# Autodesk Inventor assembly: Gearbox - 54 to 1
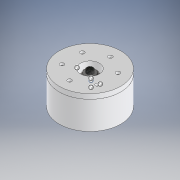
[picture p0: Inventor's stored thumbnail of the model, 180x180]
Saved by Autodesk Inventor 2017 SP1 (Build 210196100, 196)
## iProperties
Created: 2017-09-22
Part Number: Gearbox - 54 to 1
Document SubType Name: Assembly
Designer: Zach
Author: Zach
## Documents named in this file (9)
- C:\Users\Zach\Documents\GitHub\tr1\lib\Gearbox 8;1\Gearbox 8;1.iam
- C:\Users\Zach\Documents\GitHub\tr1\lib\Gearbox 8;1\Base.ipt
- C:\Users\Zach\Documents\GitHub\tr1\lib\22x8x8mm Bearing.ipt
- C:\Users\Zach\Documents\GitHub\tr1\lib\Gearbox 8;1\3mm Brass Rod.ipt
- C:\Users\Zach\Documents\GitHub\tr1\lib\CNS 3129 - M 8 x 1.25.ipt
- C:\Users\Zach\Documents\GitHub\tr1\lib\Gearbox 8;1\GearSet 1.iam
- C:\Users\Zach\Documents\GitHub\tr1\lib\Gearbox 8;1\Small Gear.ipt
- C:\Users\Zach\Documents\GitHub\tr1\lib\Gearbox 8;1\Cover.ipt
- C:\Users\Zach\Documents\Inventor\Content Center Files\R2017\en-US\ISO 4018\ISO 4018 - M8 x 40.ipt
## Components (11 placed, 7 different names)
1. Base:1 — Mate:1, Flush:1, Mate:7, Flush:5, Mate:8, Flush:6, Mate:173, Mate:179
2. ISO 4018 M8 x 40:1 — Mate:2, Mate:63, Mate:105, Mate:156, Mate:176, Mate:178, Rotation:4
3. CNS 3129 M 8:1 — Mate:105, Mate:158
4. 3mm Brass Rod:3 — Mate:8, Flush:6, Mate:172
5. 3mm Brass Rod:4 — Mate:7, Flush:5, Mate:174
6. 22x8x8mm Bearing:1 — Mate:1, Flush:1, Mate:2, Mate:63, Mate:181
7. 22x8x8mm Bearing:2 — Mate:156, Mate:158, Mate:180
8. GearSet 1:1 [sub-assembly] — Mate:172, Mate:173, Mate:175, Rotation:1, Rotation:2
9. GearSet 1:2 [sub-assembly] — Mate:174, Mate:175, Rotation:1, Rotation:3
10. Spur Gear1:1 — Mate:176, Rotation:2, Rotation:4, Mate:181
11. Spur Gear1:2 — Mate:178, Mate:179, Rotation:3, Mate:180
## Relationships (24: Mate 17, RelateRotation 4, Flush 3)
- Mate:1: Base:1 ↔ 22x8x8mm Bearing:1
- Flush:1: Base:1 ↔ 22x8x8mm Bearing:1
- Mate:2: ISO 4018 M8 x 40:1 ↔ 22x8x8mm Bearing:1
- Mate:7: Base:1 ↔ 3mm Brass Rod:4
- Flush:5: Base:1 ↔ 3mm Brass Rod:4
- Mate:8: Base:1 ↔ 3mm Brass Rod:3
- Flush:6: Base:1 ↔ 3mm Brass Rod:3
- Mate:63: ISO 4018 M8 x 40:1 ↔ 22x8x8mm Bearing:1
- Mate:105: ISO 4018 M8 x 40:1 ↔ CNS 3129 M 8:1
- Mate:156: ISO 4018 M8 x 40:1 ↔ 22x8x8mm Bearing:2
- Mate:158: CNS 3129 M 8:1 ↔ 22x8x8mm Bearing:2
- Mate:172: 3mm Brass Rod:3 ↔ GearSet 1:1
- Mate:173: Base:1 ↔ GearSet 1:1
- Mate:174: 3mm Brass Rod:4 ↔ GearSet 1:2
- Mate:175: GearSet 1:1 ↔ GearSet 1:2
- Rotation:1 [RelateRotation] (0.4815 ul): GearSet 1:1 ↔ GearSet 1:2
- Mate:176: ISO 4018 M8 x 40:1 ↔ Spur Gear1:1
- Rotation:2 [RelateRotation] (0.4815 ul): GearSet 1:1 ↔ Spur Gear1:1
- Mate:178: ISO 4018 M8 x 40:1 ↔ Spur Gear1:2
- Mate:179: Base:1 ↔ Spur Gear1:2
- Rotation:3 [RelateRotation] (0.4815 ul): GearSet 1:2 ↔ Spur Gear1:2
- Mate:180: 22x8x8mm Bearing:2 ↔ Spur Gear1:2
- Rotation:4 [RelateRotation] (1 ul): ISO 4018 M8 x 40:1 ↔ Spur Gear1:1
- Mate:181: 22x8x8mm Bearing:1 ↔ Spur Gear1:1
